# Autodesk Inventor assembly: Heatbed Assembly
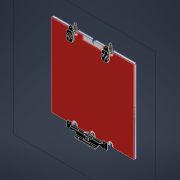
[picture p0: Inventor's stored thumbnail of the model, 180x180]
Saved by Autodesk Inventor 2022.2 (Build 262287010, 287A)
## iProperties
Created: 2022-03-13
Part Number: Heatbed Assembly
Document SubType Name: Assembly
Designer: sleib
Author: sleib
## Documents named in this file (6)
- C:\Users\sleib\Projekte\Voron-2\CAD\Inventor\Heatbed Assembly.iam
- C:\Users\sleib\Projekte\Voron-2\CAD\Inventor\Heatbed Sandwich.iam
- C:\Users\sleib\Projekte\Voron-2\CAD\Inventor\Kinematic-Mount Back.iam
- C:\Users\sleib\Projekte\Voron-2\CAD\Inventor\Kinematic-Mount Front [A].iam
- C:\Users\sleib\Projekte\Voron-2\CAD\Inventor\Kinematic-Mount Front [B].iam
- C:\Users\sleib\OneDrive\Dokumente\Inventor\Content Center Files\R2022\de-DE\DIN EN ISO 7093-2\DIN EN ISO 7093-2 - 3.ipt
## Components (7 placed, 5 different names)
1. Heatbed Sandwich:1 [sub-assembly] — Passend:1, Passend:2, Passend:3, Winkel:1, Winkel:2, Winkel:3, Passend:10, Passend:11, Passend:12, Passend:13, Passend:14, Passend:15
2. Kinematic-Mount Back:1 [sub-assembly] — Passend:1, Winkel:1, Passend:8, Passend:9
3. Kinematic-Mount Front [A]:1 [sub-assembly] — Passend:2, Winkel:2, Passend:4, Passend:5
4. Kinematic-Mount Front [B]:1 [sub-assembly] — Passend:3, Winkel:3, Passend:6, Passend:7
5. DIN EN ISO 7093-2 3:1 — Passend:4, Passend:5, Passend:12, Passend:13
6. DIN EN ISO 7093-2 3:2 — Passend:6, Passend:7, Passend:14, Passend:15
7. DIN EN ISO 7093-2 3:3 — Passend:8, Passend:9, Passend:10, Passend:11
## Relationships (18: Mate 15, Angle 3)
- Passend:1 [Mate]: Heatbed Sandwich:1 ↔ Kinematic-Mount Back:1
- Passend:2 [Mate]: Heatbed Sandwich:1 ↔ Kinematic-Mount Front [A]:1
- Passend:3 [Mate]: Heatbed Sandwich:1 ↔ Kinematic-Mount Front [B]:1
- Winkel:1 [Angle] (0 deg): Heatbed Sandwich:1 ↔ Kinematic-Mount Back:1
- Winkel:2 [Angle] (0 deg): Heatbed Sandwich:1 ↔ Kinematic-Mount Front [A]:1
- Winkel:3 [Angle] (0 deg): Heatbed Sandwich:1 ↔ Kinematic-Mount Front [B]:1
- Passend:4 [Mate]: Kinematic-Mount Front [A]:1 ↔ DIN EN ISO 7093-2 3:1
- Passend:5 [Mate]: Kinematic-Mount Front [A]:1 ↔ DIN EN ISO 7093-2 3:1
- Passend:6 [Mate]: Kinematic-Mount Front [B]:1 ↔ DIN EN ISO 7093-2 3:2
- Passend:7 [Mate]: Kinematic-Mount Front [B]:1 ↔ DIN EN ISO 7093-2 3:2
- Passend:8 [Mate]: Kinematic-Mount Back:1 ↔ DIN EN ISO 7093-2 3:3
- Passend:9 [Mate]: Kinematic-Mount Back:1 ↔ DIN EN ISO 7093-2 3:3
- Passend:10 [Mate]: Heatbed Sandwich:1 ↔ DIN EN ISO 7093-2 3:3
- Passend:11 [Mate]: Heatbed Sandwich:1 ↔ DIN EN ISO 7093-2 3:3
- Passend:12 [Mate]: Heatbed Sandwich:1 ↔ DIN EN ISO 7093-2 3:1
- Passend:13 [Mate]: Heatbed Sandwich:1 ↔ DIN EN ISO 7093-2 3:1
- Passend:14 [Mate]: Heatbed Sandwich:1 ↔ DIN EN ISO 7093-2 3:2
- Passend:15 [Mate]: Heatbed Sandwich:1 ↔ DIN EN ISO 7093-2 3:2
